# Autodesk Inventor assembly: 조립형상
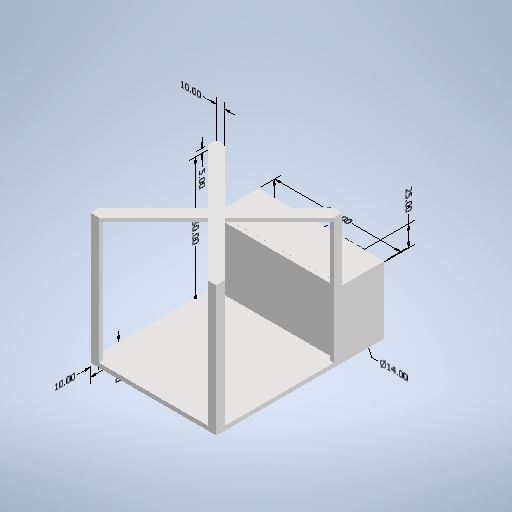
[picture p0: Inventor's stored thumbnail of the model, 512x512]
Saved by Autodesk Inventor 2025 (Build 290162000, 162)
## iProperties
Created: 2024-06-08
Part Number: 조립형상
Document SubType Name: Assembly
Designer: goomi
Author: goomi
## Documents named in this file (4)
- C:\Users\goomi\OneDrive\바탕 화면\기로공\model\조립형상.iam
- C:\Users\goomi\OneDrive\바탕 화면\기로공\model\적재부 상판.ipt
- C:\Users\goomi\OneDrive\바탕 화면\기로공\model\적재부 하판.ipt
- C:\Users\goomi\OneDrive\문서\Inventor\Content Center Files\R2025\제어부 커버.ipt
## Components (3 placed, 3 different names)
1. 적재부 상판:1 — 강체:3
2. 적재부 하판:1 — 강체:2, 강체:3
3. 제어부 커버:1 — 강체:2
## Relationships (2: WeldJoint 2)
- 강체:2 [WeldJoint]: 적재부 하판:1 ↔ 제어부 커버:1
- 강체:3 [WeldJoint]: 적재부 상판:1 ↔ 적재부 하판:1
